# Autodesk Inventor assembly: FullAssembly1
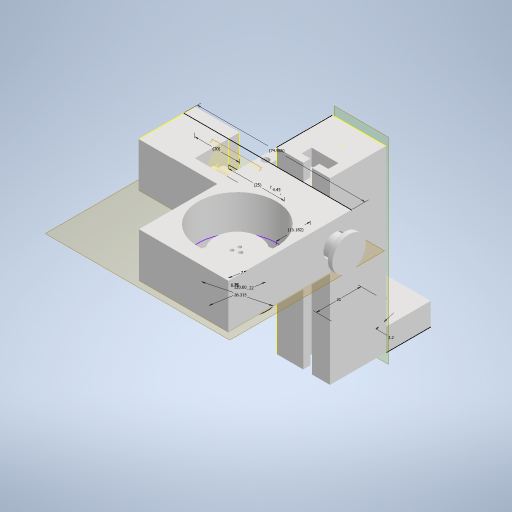
[picture p0: Inventor's stored thumbnail of the model, 512x512]
Saved by Autodesk Inventor 2023 (Build 270158000, 158)
## iProperties
Created: 2025-10-02
Part Number: FullAssembly1
Document SubType Name: Assembly
Designer: ptato_qo49uko
Author: ptato_qo49uko
## Documents named in this file (6)
- C:\Users\ptato_qo49uko\Documents\Inventor\PumpProject\Renders\FullAssembly1.iam
- C:\Users\ptato_qo49uko\Documents\Inventor\PumpProject\cap.ipt
- C:\Users\ptato_qo49uko\Documents\Inventor\PumpProject\pin.ipt
- C:\Users\ptato_qo49uko\Documents\Inventor\PumpProject\spoutextrusion.ipt
- C:\Users\ptato_qo49uko\Documents\Inventor\PumpProject\spoutstand.ipt
- C:\Users\ptato_qo49uko\Documents\Inventor\PumpProject\teethset.ipt
## Components (5 placed, 5 different names)
1. cap:1 — Mate:10, Mate:11, Mate:12
2. pin:1 — Mate:6
3. spoutextrusion:1 — Mate:3, Mate:6, Mate:7, Mate:8, Mate:9, Mate:10, Mate:11, Mate:12
4. spoutstand:1 — Mate:2, Angle:1, Mate:3
5. teethset:1 — Mate:7, Mate:8, Mate:9
## Relationships (10: Mate 9, Angle 1)
- Mate:2: spoutstand:1
- Angle:1 (0 deg): spoutstand:1
- Mate:3: spoutextrusion:1 ↔ spoutstand:1
- Mate:6: pin:1 ↔ spoutextrusion:1
- Mate:7: spoutextrusion:1 ↔ teethset:1
- Mate:8: spoutextrusion:1 ↔ teethset:1
- Mate:9: spoutextrusion:1 ↔ teethset:1
- Mate:10: cap:1 ↔ spoutextrusion:1
- Mate:11: cap:1 ↔ spoutextrusion:1
- Mate:12 (10 mm): cap:1 ↔ spoutextrusion:1
